# Autodesk Inventor assembly: FULL
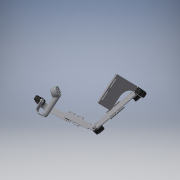
[picture p0: Inventor's stored thumbnail of the model, 180x180]
Saved by Autodesk Inventor 2019 (Build 230136000, 136)
## iProperties
Created: 2018-10-22
Part Number: FULL
Material: 일반
Document SubType Name: Assembly
Designer: otm09
Author: otm09
## Documents named in this file (9)
- D:\User\project\3D\bizcol\FULL.iam
- D:\User\project\3D\bizcol\arm1.ipt
- D:\User\project\3D\bizcol\AX-12A\AX-12.iam
- D:\User\project\3D\bizcol\shoulder1.ipt
- D:\User\project\3D\bizcol\shoulder2.ipt
- D:\User\project\3D\bizcol\hand_joy.ipt
- D:\User\project\3D\bizcol\hand_joy_cover.ipt
- D:\User\project\3D\bizcol\hand.ipt
- D:\User\project\3D\bizcol\hand-1.ipt
## Components (12 placed, 8 different names)
1. arm1:1 — 강체:2, 강체:7
2. AX-12:1 [sub-assembly] — 강체:7, 회전:7
3. shoulder1:1 — 강체:8
4. AX-12:2 [sub-assembly] — 강체:8, 회전:3
5. arm1:2 — 강체:1, 강체:2
6. shoulder2:1 — 회전:3, 회전:4
7. AX-12:3 [sub-assembly] — 회전:4, 강체:1
8. hand_joy:1 — 회전:6, 강체:11
9. hand_joy_cover:1 — 강체:11
10. AX-12:4 [sub-assembly] — 회전:6, 강체:14
11. hand:1 — 강체:12, 회전:7
12. hand-1:1 — 강체:12, 강체:14
## Relationships (11: WeldJoint 7, RevoluteJoint 4)
- 강체:8 [WeldJoint]: shoulder1:1 ↔ AX-12:2
- 회전:3 [RevoluteJoint]: AX-12:2 ↔ shoulder2:1
- 회전:4 [RevoluteJoint]: shoulder2:1 ↔ AX-12:3
- 강체:1 [WeldJoint]: arm1:2 ↔ AX-12:3
- 강체:2 [WeldJoint]: arm1:1 ↔ arm1:2
- 강체:7 [WeldJoint]: arm1:1 ↔ AX-12:1
- 회전:6 [RevoluteJoint]: hand_joy:1 ↔ AX-12:4
- 강체:11 [WeldJoint]: hand_joy:1 ↔ hand_joy_cover:1
- 강체:12 [WeldJoint]: hand:1 ↔ hand-1:1
- 강체:14 [WeldJoint]: AX-12:4 ↔ hand-1:1
- 회전:7 [RevoluteJoint]: AX-12:1 ↔ hand:1
